# Autodesk Inventor assembly: FLUGGER REGULATOR ASSY
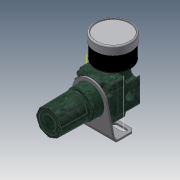
[picture p0: Inventor's stored thumbnail of the model, 180x180]
Saved by Autodesk Inventor 2020.3 (Build 243373000, 373)
## iProperties
RuleStatus: InUse
AfterDocSave0: file://Part Number Cleaner
Created: 2015-05-13
Vendor: HHMI: JRC - ID&F
Document SubType Name: Assembly
Designer: ARNOLDJ
Description: REGULATOR AND GAUGE ASSY
DESIGN DEPARTMENT: HHMI: JRC - ID&F
ALTERED ITEM PART NUMBER: N/A
ALTERED ITEM VENDOR: N/A
ALTERED ITEM DESCRIPTION: N/A
Author: ARNOLDJ
Revision Number: 0
## Documents named in this file (4)
- C:\_WORKSPACE\DATA\PROJECTS\_PROJECTS BY LAB\CARD (LAB)\FLUGGER\FLUGGER REGULATOR ASSY.iam
- C:\_WORKSPACE\DATA\COMMON\Clippard\MMR-2P.ipt
- C:\_WORKSPACE\DATA\COMMON\Clippard\MMH-B220.ipt
- C:\_WORKSPACE\DATA\COMMON\Clippard\CLIPPARD PG-15-60P.ipt
## Components (3 placed, 3 different names)
1. MMR-2P:1 — Mate:1, Mate:2, Mate:5, Mate:6
2. MMH-B220:1 — Mate:1, Mate:2, Angle:1
3. CLIPPARD PG-15-60P:1 — Mate:5, Mate:6
## Relationships (5: Mate 4, Angle 1)
- Mate:1: MMR-2P:1 ↔ MMH-B220:1
- Mate:2: MMR-2P:1 ↔ MMH-B220:1
- Angle:1 (180 deg): MMH-B220:1
- Mate:5 (6.35 mm): MMR-2P:1 ↔ CLIPPARD PG-15-60P:1
- Mate:6: MMR-2P:1 ↔ CLIPPARD PG-15-60P:1
